# Autodesk Inventor assembly: przegub_6
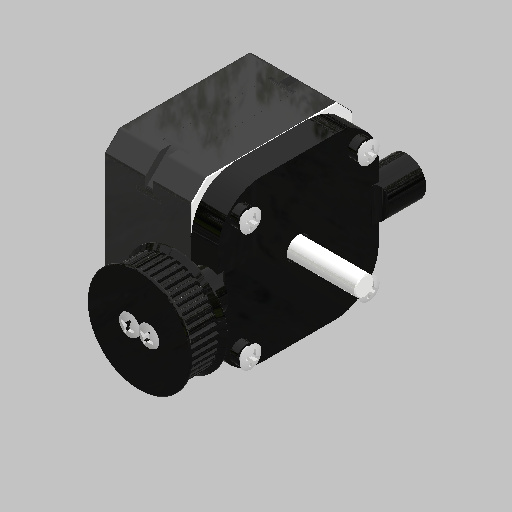
[picture p0: Inventor's stored thumbnail of the model, 512x512]
Saved by Autodesk Inventor 2024.3 (Build 283343000, 343)
## iProperties
Created: 2025-10-11
Part Number: przegub_6
Document SubType Name: Assembly
Designer: User
Mass: 53.1781 g
Surface Area: 320.123 cm^2
Volume: 53.1781 cm^3
Density: 1 g/cm^3
Author: User
## Documents named in this file (6)
- C:\Users\Duszy\Desktop\Dummy_v2\Model\Model\przegub_6\przegub_6.iam
- C:\Users\Duszy\Desktop\Dummy_v2\Model\Model\przegub_6\94459A769_Heat-Set Inserts for Plastic.ipt
- C:\Users\Duszy\Desktop\Dummy_v2\Model\Model\przegub_6\Component1.ipt
- C:\Users\Duszy\Desktop\Dummy_v2\Model\Model\przegub_6\end_efector_2.ipt
- C:\Users\Duszy\Desktop\Dummy_v2\Model\Model z feedback\przegub_3\m3-10mm.ipt
- C:\Users\Duszy\Desktop\Dummy_v2\Model\Model\przegub_6\NEMA 17 Stepper Motor 23mm-NEMA 17 Stepper Motor 23mm.ipt
## Components (11 placed, 5 different names)
1. Component1:1 — Sztywne:3
2. end_efector_2:1 — Sztywne:3, Sztywne:4, Sztywne:5, Sztywne:6, Obrotowe:1, Obrotowe:2, Obrotowe:3
3. NEMA 17 Stepper Motor 23mm-NEMA 17 Stepper Motor 23mm:1 — Sztywne:4
4. 94459A769_Heat-Set Inserts for Plastic:3 — Sztywne:5
5. m3-10mm:3 — Sztywne:6
6. 94459A769_Heat-Set Inserts for Plastic:4 — Obrotowe:1
7. m3-10mm:4 — Obrotowe:2
8. m3-10mm:5 — Obrotowe:3
9. m3-10mm:6
10. m3-10mm:7
11. m3-10mm:8
## Component patterns: (4 elements, first: m3-10mm:5)
## Relationships (7: WeldJoint 4, RevoluteJoint 3)
- Sztywne:3 [WeldJoint]: Component1:1 ↔ end_efector_2:1
- Sztywne:4 [WeldJoint]: end_efector_2:1 ↔ NEMA 17 Stepper Motor 23mm-NEMA 17 Stepper Motor 23mm:1
- Sztywne:5 [WeldJoint]: end_efector_2:1 ↔ 94459A769_Heat-Set Inserts for Plastic:3
- Sztywne:6 [WeldJoint]: end_efector_2:1 ↔ m3-10mm:3
- Obrotowe:1 [RevoluteJoint]: end_efector_2:1 ↔ 94459A769_Heat-Set Inserts for Plastic:4
- Obrotowe:2 [RevoluteJoint]: end_efector_2:1 ↔ m3-10mm:4
- Obrotowe:3 [RevoluteJoint] (9 mm): end_efector_2:1 ↔ m3-10mm:5
